# Autodesk Inventor assembly: писюны
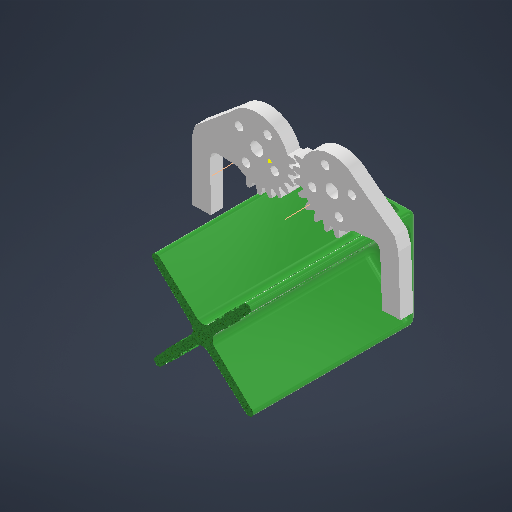
[picture p0: Inventor's stored thumbnail of the model, 512x512]
Saved by Autodesk Inventor 2025 (Build 290162000, 162)
## iProperties
Created: 2024-12-28
Part Number: писюны
Document SubType Name: Assembly
Designer: Phantom
Author: Phantom
## Documents named in this file (5)
- C:\Users\GameHD\Desktop\phantom 16950\писюны.iam
- C:\Users\GameHD\Desktop\phantom 16950\am-5401 Sample.ipt
- C:\Users\GameHD\Desktop\phantom 16950\писюн.ipt
- C:\Users\GameHD\Desktop\phantom 16950\писюн 2.ipt
- C:\Users\GameHD\Downloads\Telegram Desktop\Клешни с фиксатором\Клешни с фиксатором.ipt
## Components (6 placed, 4 different names)
1. am-5401 Sample:1
2. Клешни с фиксатором:4
3. писюн 2:1
4. писюн:1
5. писюн 2:2 — Совмещение:1, Заподлицо:1
6. писюн:2 — Совмещение:2, Заподлицо:1
## Relationships (3: Mate 2, Flush 1)
- Совмещение:1 [Mate]: писюн 2:2
- Совмещение:2 [Mate]: писюн:2
- Заподлицо:1 [Flush]: писюн 2:2 ↔ писюн:2
